# Autodesk Inventor assembly: Assembly1
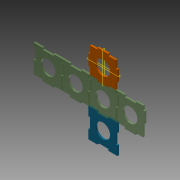
[picture p0: Inventor's stored thumbnail of the model, 180x180]
Saved by Autodesk Inventor 2014 SP2 (Build 180246200, 246)
## iProperties
Created: 2014-11-21
Part Number: Assembly1
Document SubType Name: Assembly
Designer: JLM
Author: JLM
## Documents named in this file (4)
- C:\Users\JLM\Documents\Art\Puzzle Box\ASizeBox\ABox Assem.iam
- C:\Users\JLM\Documents\Art\Puzzle Box\ASizeBox\ASide.ipt
- C:\Users\JLM\Documents\Art\Puzzle Box\ASizeBox\ATop.ipt
- C:\Users\JLM\Documents\Art\Puzzle Box\ASizeBox\ABottom.ipt
## Components (6 placed, 3 different names)
1. ASide:1 — Mate:5, Flush:4, Flush:5, Mate:6, Flush:6, Flush:8, Flush:9, Flush:11, Flush:12, Mate:7, Mate:8
2. ATop:1 — Mate:6, Flush:6
3. ABottom:1 — Mate:5, Flush:4, Flush:5
4. ASide:2 — Flush:7, Flush:8, Flush:10, Flush:11, Mate:8, Mate:9
5. ASide:3 — Flush:7, Flush:10, Mate:9
6. ASide:4 — Flush:9, Flush:12, Mate:7
## Relationships (14: Flush 9, Mate 5)
- Mate:5: ASide:1 ↔ ABottom:1
- Flush:4: ASide:1 ↔ ABottom:1
- Flush:5: ASide:1 ↔ ABottom:1
- Mate:6: ASide:1 ↔ ATop:1
- Flush:6: ASide:1 ↔ ATop:1
- Flush:7: ASide:2 ↔ ASide:3
- Flush:8: ASide:1 ↔ ASide:2
- Flush:9: ASide:1 ↔ ASide:4
- Flush:10: ASide:2 ↔ ASide:3
- Flush:11: ASide:1 ↔ ASide:2
- Flush:12: ASide:1 ↔ ASide:4
- Mate:7: ASide:1 ↔ ASide:4
- Mate:8: ASide:1 ↔ ASide:2
- Mate:9: ASide:2 ↔ ASide:3
